# Autodesk Inventor assembly: Сборка3
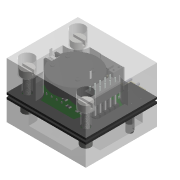
[picture p0: Inventor's stored thumbnail of the model, 180x180]
Saved by Autodesk Inventor 2015 SP1 (Build 190203100, 203)
## iProperties
Created: 2015-12-01
Part Number: Сборка3
Document SubType Name: Assembly
Designer: User
Mass: 32.1815 g
Surface Area: 211.427 cm^2
Volume: 23.2526 cm^3
Density: 1.38399 g/cm^3
Author: User
Title: external
## Documents named in this file (14)
- C:\Users\User\Downloads\kurs_mark\Inventor\Сборка3.iam
- C:\Users\User\Downloads\kurs_mark\Inventor\conn_sensor.ipt
- C:\Users\User\Downloads\kurs_mark\Inventor\button.ipt
- C:\Users\User\Downloads\kurs_mark\Inventor\Imported Components\fuel_level_1h2\fuel_level_1h2.iam
- C:\Users\User\Downloads\kurs_mark\Inventor\case_top.ipt
- C:\Users\User\Downloads\kurs_mark\Inventor\bs-7.ipt
- C:\Users\User\Downloads\kurs_mark\Inventor\hdr-2x5t_2.54x2.54_13x5.ipt
- C:\Users\User\Downloads\kurs_mark\Inventor\MOLEX.ipt
- C:\Users\User\Downloads\kurs_mark\Inventor\jumper.ipt
- C:\Users\User\Downloads\kurs_mark\Inventor\case_bottom.ipt
- C:\Users\User\Downloads\kurs_mark\Inventor\resin_bottom.ipt
- C:\Users\User\Downloads\kurs_mark\Inventor\resin_top.ipt
- C:\Users\User\Downloads\kurs_mark\Inventor\bonka.ipt
- C:\Users\User\Downloads\kurs_mark\Inventor\screw_M3-16.ipt
## Components (17 placed, 13 different names)
1. conn_sensor:1 — Жесткий:2
2. button:1 — Жесткий:3
3. fuel_level_1h2:1 [sub-assembly] — Жесткий:2, Жесткий:3, Заподлицо:3, Заподлицо:4
4. case_top:1 — Цилиндрический:1, Жесткий:6, Rigid:7, Rigid:8, Rigid:9
5. bs-7:1 — Совмещение:1
6. hdr-2x5t_2.54x2.54_13x5:1
7. MOLEX:1 — Совмещение:1, Заподлицо:4, Заподлицо:5, Совмещение:2
8. jumper:1 — Заподлицо:5
9. case_bottom:1 — Совмещение:2, Цилиндрический:1, Rigid:10, Rigid:11, Rigid:12
10. resin_bottom:1
11. resin_top:1 — Жесткий:6
12. bonka:1 — Rigid:7
13. bonka:2 — Rigid:8
14. bonka:3 — Rigid:9
15. screw_M3-16:1 — Rigid:12
16. screw_M3-16:2 — Rigid:11
17. screw_M3-16:3 — Rigid:10
## Relationships (15: WeldJoint 9, Flush 3, Mate 2, CylindricalJoint 1)
- Жесткий:2 [WeldJoint] (0.3 mm): conn_sensor:1 ↔ fuel_level_1h2:1
- Жесткий:3 [WeldJoint]: button:1 ↔ fuel_level_1h2:1
- Совмещение:1 [Mate]: bs-7:1 ↔ MOLEX:1
- Заподлицо:3 [Flush]: fuel_level_1h2:1
- Заподлицо:4 [Flush] (-11 mm): fuel_level_1h2:1 ↔ MOLEX:1
- Заподлицо:5 [Flush]: MOLEX:1 ↔ jumper:1
- Совмещение:2 [Mate]: MOLEX:1 ↔ case_bottom:1
- Цилиндрический:1 [CylindricalJoint]: case_top:1 ↔ case_bottom:1
- Жесткий:6 [WeldJoint]: case_top:1 ↔ resin_top:1
- Rigid:7 [WeldJoint]: case_top:1 ↔ bonka:1
- Rigid:8 [WeldJoint]: case_top:1 ↔ bonka:2
- Rigid:9 [WeldJoint]: case_top:1 ↔ bonka:3
- Rigid:10 [WeldJoint]: case_bottom:1 ↔ screw_M3-16:3
- Rigid:11 [WeldJoint]: case_bottom:1 ↔ screw_M3-16:2
- Rigid:12 [WeldJoint]: case_bottom:1 ↔ screw_M3-16:1
